# Autodesk Inventor assembly: ElectronicsAssembly
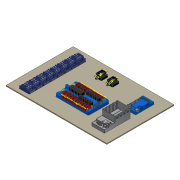
[picture p0: Inventor's stored thumbnail of the model, 180x180]
Saved by Autodesk Inventor 2012 (Build 160160000, 160)
## iProperties
Created: 2013-01-30
Part Number: ElectronicsAssembly
Document SubType Name: Assembly
Designer: JesseK
Mass: 2725.39 g
Surface Area: 16081.3 cm^2
Volume: 3257.05 cm^3
Density: 0.836766 g/cm^3
Author: JesseK
## Documents named in this file (7)
- Z:\UserData\Documents\Inventor\team1885frc\Robot2013\Electronics\ElectronicsAssembly.iam
- Z:\UserData\Documents\Inventor\team1885frc\Robot2013\Electronics\ElectronicsBoard.ipt
- Z:\UserData\Documents\Inventor\team1885frc\Electronics\spike relay\Spike_Assem.iam
- Z:\UserData\Documents\Inventor\team1885frc\Electronics\PowerDistributionBoard\elc_Power_Distro_inv.iam
- Z:\UserData\Documents\Inventor\team1885frc\Electronics\cRIO_4Slot\Imported Components\cu_crio-9075_4-slot\cu_crio-9075_4-slot.ipt
- Z:\UserData\Documents\Inventor\team1885frc\Electronics\DigitalSidecar\elc_Digital_Sidecar_inv.iam
- Z:\UserData\Documents\Inventor\team1885frc\AndyMark\Talon.ipt
## Components (14 placed, 6 different names)
1. ElectronicsBoard:1 — Mate:1, Mate:2, Flush:1, Mate:3, Mate:4, Flush:2, Mate:6, Mate:7, Mate:8, Mate:9, Mate:10, Mate:11, Mate:12, Mate:13, Mate:14, Mate:15, Mate:30
2. Spike_Assem:1 [sub-assembly] — Mate:4, Flush:3, Mate:5
3. Spike_Assem:2 [sub-assembly] — Mate:3, Flush:2, Flush:3, Mate:5
4. elc_Power_Distro_inv:1 [sub-assembly] — Mate:6
5. cu_crio-9075_4-slot:1 — Mate:1
6. elc_Digital_Sidecar_inv:1 [sub-assembly] — Mate:2, Flush:1
7. Talon:1 — Mate:13, Mate:16, Mate:17, Mate:18, Mate:19
8. Talon:2 — Mate:12, Mate:17, Mate:19, Mate:20, Mate:25
9. Talon:3 — Mate:8, Mate:24, Mate:29
10. Talon:4 — Mate:7, Mate:22, Mate:23, Mate:27, Mate:28
11. Talon:5 — Mate:10, Mate:20, Mate:21, Mate:25, Mate:26
12. Talon:6 — Mate:14, Mate:15, Mate:16, Mate:18, Mate:30
13. Talon:7 — Mate:11, Mate:21, Mate:22, Mate:26, Mate:27
14. Talon:8 — Mate:9, Mate:23, Mate:24, Mate:28, Mate:29
## Relationships (33: Mate 30, Flush 3)
- Mate:1: ElectronicsBoard:1 ↔ cu_crio-9075_4-slot:1
- Mate:2: ElectronicsBoard:1 ↔ elc_Digital_Sidecar_inv:1
- Flush:1 (76.2 mm): ElectronicsBoard:1 ↔ elc_Digital_Sidecar_inv:1
- Mate:3: ElectronicsBoard:1 ↔ Spike_Assem:2
- Mate:4: ElectronicsBoard:1 ↔ Spike_Assem:1
- Flush:2 (50.8 mm): ElectronicsBoard:1 ↔ Spike_Assem:2
- Flush:3: Spike_Assem:1 ↔ Spike_Assem:2
- Mate:5 (76.2 mm): Spike_Assem:1 ↔ Spike_Assem:2
- Mate:6: ElectronicsBoard:1 ↔ elc_Power_Distro_inv:1
- Mate:7: ElectronicsBoard:1 ↔ Talon:4
- Mate:8: ElectronicsBoard:1 ↔ Talon:3
- Mate:9: ElectronicsBoard:1 ↔ Talon:8
- Mate:10: ElectronicsBoard:1 ↔ Talon:5
- Mate:11: ElectronicsBoard:1 ↔ Talon:7
- Mate:12: ElectronicsBoard:1 ↔ Talon:2
- Mate:13: ElectronicsBoard:1 ↔ Talon:1
- Mate:14: ElectronicsBoard:1 ↔ Talon:6
- Mate:15 (-25.4 mm): ElectronicsBoard:1 ↔ Talon:6
- Mate:16: Talon:1 ↔ Talon:6
- Mate:17: Talon:1 ↔ Talon:2
- Mate:18: Talon:1 ↔ Talon:6
- Mate:19: Talon:1 ↔ Talon:2
- Mate:20: Talon:2 ↔ Talon:5
- Mate:21: Talon:5 ↔ Talon:7
- Mate:22: Talon:4 ↔ Talon:7
- Mate:23: Talon:4 ↔ Talon:8
- Mate:24: Talon:3 ↔ Talon:8
- Mate:25: Talon:2 ↔ Talon:5
- Mate:26: Talon:5 ↔ Talon:7
- Mate:27: Talon:4 ↔ Talon:7
- Mate:28: Talon:4 ↔ Talon:8
- Mate:29: Talon:3 ↔ Talon:8
- Mate:30 (-63.5 mm): ElectronicsBoard:1 ↔ Talon:6
